# Autodesk Inventor assembly: Suspension
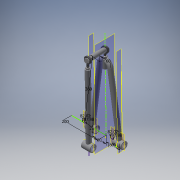
[picture p0: Inventor's stored thumbnail of the model, 180x180]
Saved by Autodesk Inventor 2016 SP1 (Build 200210100, 210)
## iProperties
Created: 2016-06-15
Part Number: Suspension
Document SubType Name: Assembly
Designer: asvsf
Author: asvsf
## Documents named in this file (10)
- C:\Project\Buggy\Suspension\Suspension.iam
- C:\Project\Buggy\Suspension\upper_arm.iam
- C:\Project\Carv2\Carv2\Carv2\lower_arm.iam
- C:\Project\Buggy\Suspension\SA12E\SA 12 E.ipt
- C:\Users\asvsf\Documents\Inventor\Content Center Files\R2016\en-US\ISO 4032(1)\ISO 4032 - M12DIN EN.ipt
- C:\Project\Buggy\Suspension\amrs_link.iam
- C:\Users\asvsf\Documents\Inventor\Content Center Files\R2016\en-US\DIN EN 14399-4(1)\DIN EN 14399-4 - M12 x 45.ipt
- C:\Project\Buggy\Suspension\upper_arm\Design Accelerator\Bearing1.iam
- C:\Project\Buggy\Suspension\upper_arm_004.ipt
- C:\Project\Buggy\Suspension\arm_borne.iam
## Components (16 placed, 9 different names)
1. upper_arm:1 [sub-assembly] — Angle:1, Mate:2, Mate:4, Mate:5, Mate:8, Mate:23, Angle:2, Angle:3, Mate:26, Mate:35, Mate:36, Mate:37, Mate:38
2. lower_arm:1 [sub-assembly] — Angle:1, Mate:3, Mate:6, Mate:7, Mate:9, Angle:3, Mate:26, Flush:1, Mate:40, Mate:41
3. SA 12 E:1 — Mate:8, Mate:19, Mate:27, Mate:31, Mate:32
4. SA 12 E:2 — Mate:9, Mate:22, Mate:28, Mate:30
5. DIN EN 24032 M12:1 — Mate:6, Mate:7, Mate:22
6. DIN EN 24032 M12:2 — Mate:4, Mate:5, Mate:19
7. amrs_link:1 [sub-assembly] — Mate:10, Mate:11, Mate:20, Mate:21, Mate:29, Mate:32
8. DIN EN 24032 M12:3 — Mate:10, Mate:11, Mate:15
9. DIN EN 24032 M12:4 — Mate:20, Mate:21
10. DIN EN 14399-4 M12 x 45:1 — Mate:15, Mate:27, Mate:31
11. DIN EN 14399-4 M12 x 45:2 — Mate:28, Mate:29, Mate:30
12. Bearing:1 [sub-assembly] — Flush:3, Mate:34
13. Bearing:2 [sub-assembly] — Flush:2, Mate:33
14. upper_arm_004:1 — Flush:2, Mate:33, Flush:3, Mate:34, Mate:35, Mate:36
15. upper_arm_004:2 — Mate:37, Mate:38
16. arm_borne:1 [sub-assembly] — Mate:40, Mate:41
## Relationships (38: Mate 32, Angle 3, Flush 3)
- Angle:1 (0 deg): upper_arm:1 ↔ lower_arm:1
- Mate:2: upper_arm:1
- Mate:3: lower_arm:1
- Mate:4: upper_arm:1 ↔ DIN EN 24032 M12:2
- Mate:5: upper_arm:1 ↔ DIN EN 24032 M12:2
- Mate:6: lower_arm:1 ↔ DIN EN 24032 M12:1
- Mate:7: lower_arm:1 ↔ DIN EN 24032 M12:1
- Mate:8: upper_arm:1 ↔ SA 12 E:1
- Mate:9: lower_arm:1 ↔ SA 12 E:2
- Mate:10: amrs_link:1 ↔ DIN EN 24032 M12:3
- Mate:11: amrs_link:1 ↔ DIN EN 24032 M12:3
- Mate:15: DIN EN 24032 M12:3 ↔ DIN EN 14399-4 M12 x 45:1
- Mate:19 (30 mm): SA 12 E:1 ↔ DIN EN 24032 M12:2
- Mate:20: amrs_link:1 ↔ DIN EN 24032 M12:4
- Mate:21: amrs_link:1 ↔ DIN EN 24032 M12:4
- Mate:22 (35 mm): SA 12 E:2 ↔ DIN EN 24032 M12:1
- Mate:23: upper_arm:1
- Angle:2 (0 deg): upper_arm:1
- Mate:25
- Angle:3 (0 deg): upper_arm:1 ↔ lower_arm:1
- Mate:26 (116 mm): upper_arm:1 ↔ lower_arm:1
- Flush:1 (25 mm): lower_arm:1
- Mate:27: SA 12 E:1 ↔ DIN EN 14399-4 M12 x 45:1
- Mate:28: SA 12 E:2 ↔ DIN EN 14399-4 M12 x 45:2
- Mate:29: amrs_link:1 ↔ DIN EN 14399-4 M12 x 45:2
- Mate:30: SA 12 E:2 ↔ DIN EN 14399-4 M12 x 45:2
- Mate:31: SA 12 E:1 ↔ DIN EN 14399-4 M12 x 45:1
- Mate:32: SA 12 E:1 ↔ amrs_link:1
- Flush:2: Bearing:2 ↔ upper_arm_004:1
- Mate:33: Bearing:2 ↔ upper_arm_004:1
- Flush:3: Bearing:1 ↔ upper_arm_004:1
- Mate:34: Bearing:1 ↔ upper_arm_004:1
- Mate:35: upper_arm:1 ↔ upper_arm_004:1
- Mate:36: upper_arm:1 ↔ upper_arm_004:1
- Mate:37: upper_arm:1 ↔ upper_arm_004:2
- Mate:38: upper_arm:1 ↔ upper_arm_004:2
- Mate:40: lower_arm:1 ↔ arm_borne:1
- Mate:41: lower_arm:1 ↔ arm_borne:1
